# Autodesk Inventor assembly: PlateRail24in
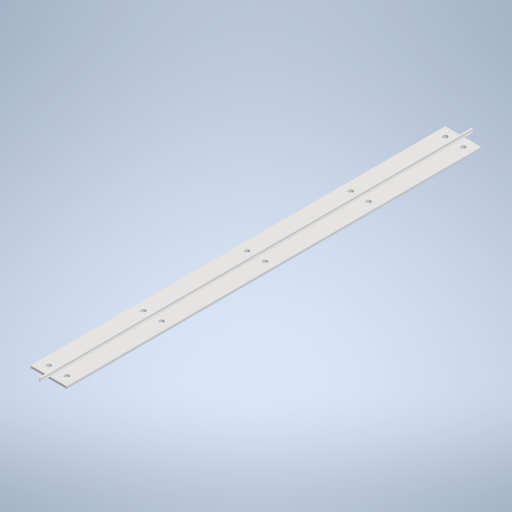
[picture p0: Inventor's stored thumbnail of the model, 512x512]
Saved by Autodesk Inventor 2023 (Build 270158030, 158C)
## iProperties
Created: 2023-02-14
Part Number: PlateRail24in
Document SubType Name: Assembly
Designer: jeremyy
Author: jeremyy
## Documents named in this file (3)
- \\andrew.ad.cmu.edu\users\users1\jeremyy\Documents\Inventor\CMU Bridge\New folder\PlateRail24in.iam
- \\andrew.ad.cmu.edu\users\users1\jeremyy\Documents\Inventor\CMU Bridge\New folder\Plate2inx23in.ipt
- \\andrew.ad.cmu.edu\users\users1\jeremyy\Documents\Inventor\CMU Bridge\New folder\Rail24in.ipt
## Components (2 placed, 2 different names)
1. Plate2inx23in:1 — Mate:1, Flush:1, Flush:2
2. Rail24in:1 — Mate:1, Flush:1, Flush:2
## Relationships (3: Flush 2, Mate 1)
- Mate:1: Plate2inx23in:1 ↔ Rail24in:1
- Flush:1 (-12.7 mm): Plate2inx23in:1 ↔ Rail24in:1
- Flush:2 (23.5458 mm): Plate2inx23in:1 ↔ Rail24in:1
